# Autodesk Inventor assembly: 組合1
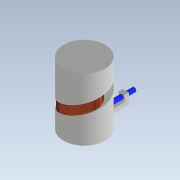
[picture p0: Inventor's stored thumbnail of the model, 180x180]
Saved by Autodesk Inventor 2022 (Build 260153000, 153)
## iProperties
Created: 2023-04-20
Part Number: 組合1
Document SubType Name: Assembly
Designer: Johnny Jou
Author: Johnny Jou
## Documents named in this file (5)
- C:\Users\Johnny Jou\Documents\GitHub\Special-project\test\組合1.iam
- C:\Users\Johnny Jou\Documents\GitHub\Special-project\CamSimulaiton\從動桿.ipt
- C:\Users\Johnny Jou\Documents\GitHub\Special-project\CamSimulaiton\滾輪.ipt
- C:\Users\Johnny Jou\Documents\GitHub\Special-project\test\零件2.ipt
- C:\Users\Johnny Jou\Documents\GitHub\Special-project\test\零件1.ipt
## Components (4 placed, 4 different names)
1. 零件2:1 — 貼合:1, 貼合:2, 角度:1
2. 零件1:1 — 貼合:1, 相切:1
3. 從動桿:1 — 插入:1, 貼合:2
4. 滾輪:1 — 插入:1, 角度:1, 相切:1
## Relationships (5: Mate 2, Insert 1, Angle 1, Tangent 1)
- 貼合:1 [Mate]: 零件2:1 ↔ 零件1:1
- 插入:1 [Insert]: 從動桿:1 ↔ 滾輪:1
- 貼合:2 [Mate]: 零件2:1 ↔ 從動桿:1
- 角度:1 [Angle] (0 deg): 零件2:1 ↔ 滾輪:1
- 相切:1 [Tangent]: 零件1:1 ↔ 滾輪:1
